# Autodesk Inventor assembly: midroller
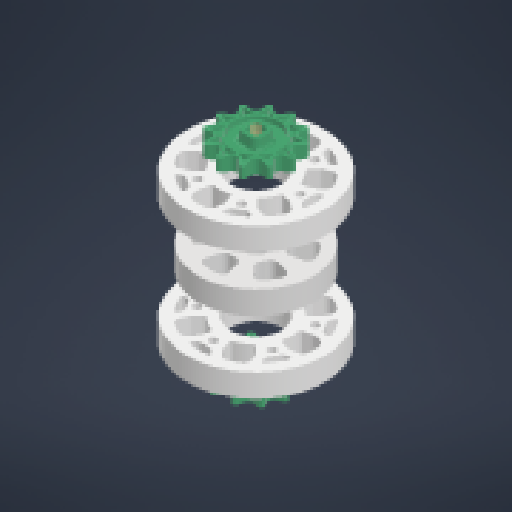
[picture p0: Inventor's stored thumbnail of the model, 512x512]
Saved by Autodesk Inventor 2025.2 (Build 292293000, 293)
## iProperties
Created: 2025-12-04
Part Number: midroller
Document SubType Name: Assembly
Designer: cloudy
Author: cloudy
## Documents named in this file (6)
- C:\Users\cloudy\Documents\GitHub\aura-cad\15\midroller.iam
- C:\Users\cloudy\Documents\GitHub\aura-cad\!lib\Motion\Wheels\Flex Wheels\3.000 Flex Wheel.ipt
- C:\Users\cloudy\Documents\GitHub\aura-cad\!lib\Motion\Sprockets\9P Sprocket\9P 12T Sprocket, No Insert.iam
- C:\Users\cloudy\Documents\GitHub\aura-cad\!lib\Motion\Sprockets\9P Sprocket.iam
- C:\Users\cloudy\Documents\GitHub\aura-cad\!lib\Motion\Wheels\Flex Wheels\3.000 Flex Wheel\3.000 30A .500.ipt
- C:\Users\cloudy\Documents\GitHub\aura-cad\15\2.5in flex.ipt
## Components (5 placed, 3 different names)
1. 3.000 30A .500:1 — Insert:1, Insert:8
2. 3.000 30A .500:2 — Insert:1, Insert:7, Insert:9
3. 2.5in flex:1 — Insert:7
4. 9P 12T Sprocket, No Insert:1 [sub-assembly] — Insert:8
5. 9P 12T Sprocket, No Insert:2 [sub-assembly] — Insert:9
## Relationships (4: Insert 4)
- Insert:1 (57.15 mm): 3.000 30A .500:1 ↔ 3.000 30A .500:2
- Insert:7 (22.225 mm): 3.000 30A .500:2 ↔ 2.5in flex:1
- Insert:8 (6.35 mm): 3.000 30A .500:1 ↔ 9P 12T Sprocket, No Insert:1
- Insert:9 (6.35 mm): 3.000 30A .500:2 ↔ 9P 12T Sprocket, No Insert:2
